# Autodesk Inventor assembly: head_fin1
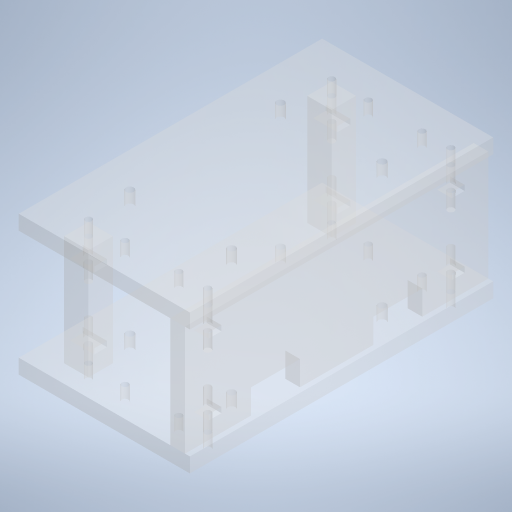
[picture p0: Inventor's stored thumbnail of the model, 512x512]
Saved by Autodesk Inventor 2024 (Build 280153000, 153)
## iProperties
Created: 2024-09-14
Part Number: head_fin1
Document SubType Name: Assembly
Designer: jmha0
Author: jmha0
## Documents named in this file (4)
- C:\Users\jmha0\OneDrive\바탕 화면\19th_intern_hjm_fight_robot\Upper_Body\head\head_fin1.iam
- C:\Users\jmha0\OneDrive\바탕 화면\19th_intern_hjm_fight_robot\Upper_Body\head\frame_head1.ipt
- C:\Users\jmha0\OneDrive\바탕 화면\19th_intern_hjm_fight_robot\Upper_Body\head\frame_head2.ipt
- C:\Users\jmha0\OneDrive\바탕 화면\19th_intern_hjm_fight_robot\Upper_Body\head\frame_head3.ipt
## Components (5 placed, 3 different names)
1. frame_head1:1 — 삽입:1, 삽입:2, 삽입:6, 삽입:8
2. frame_head2:1 — 삽입:2, 삽입:3
3. frame_head2:2 — 삽입:1, 삽입:4
4. frame_head1:2 — 삽입:3, 삽입:4, 삽입:5, 삽입:7
5. frame_head3:1 — 삽입:5, 삽입:6, 삽입:7, 삽입:8
## Relationships (8: Insert 8)
- 삽입:1 [Insert]: frame_head1:1 ↔ frame_head2:2
- 삽입:2 [Insert]: frame_head1:1 ↔ frame_head2:1
- 삽입:3 [Insert]: frame_head2:1 ↔ frame_head1:2
- 삽입:4 [Insert]: frame_head2:2 ↔ frame_head1:2
- 삽입:5 [Insert]: frame_head1:2 ↔ frame_head3:1
- 삽입:6 [Insert]: frame_head1:1 ↔ frame_head3:1
- 삽입:7 [Insert]: frame_head1:2 ↔ frame_head3:1
- 삽입:8 [Insert]: frame_head1:1 ↔ frame_head3:1
